# Autodesk Inventor assembly: 450LinearStage
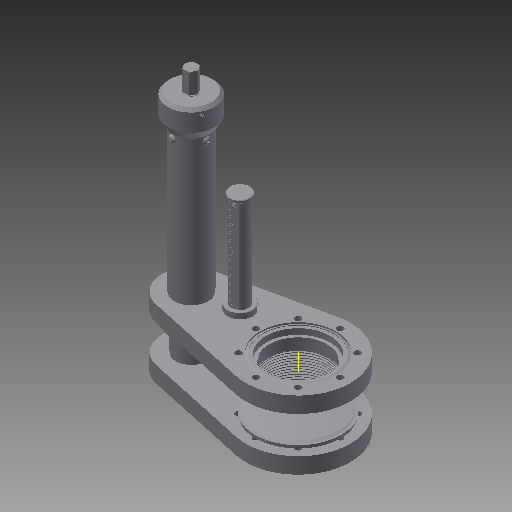
[picture p0: Inventor's stored thumbnail of the model, 512x512]
Saved by Autodesk Inventor 2018.1 (Build 221171000, 171)
## iProperties
Created: 2012-09-26
Part Number: 450LinearStage
Document SubType Name: Assembly
Designer: Sergey
Translation Standard: STEP AP203
FileName: 665524.STEP
PreProcessor: SolidWorks 2010
PostProcessor: Build: 236a, Release: 2009 RTM - Date: Fri 02/22/2008
Sent Units: Inches
Uncertainty: 1e-05
Author: Sergey
## Documents named in this file (23)
- C:\Users\michaels\Documents\SVN@Inventor\Moore Scienta DA30 system\450LinearStage.iam
- C:\Users\michaels\Documents\SVN@Inventor\Moore Scienta DA30 system\990985-04 Rev C-1-solid1.ipt
- C:\Users\michaels\Documents\SVN@Inventor\Moore Scienta DA30 system\990986-04 Rev B-1-solid1.ipt
- C:\Users\michaels\Documents\SVN@Inventor\Moore Scienta DA30 system\967848 Rev B-1-solid1.ipt
- C:\Users\michaels\Documents\SVN@Inventor\Moore Scienta DA30 system\966780 Rev --1-solid1.ipt
- C:\Users\michaels\Documents\SVN@Inventor\Moore Scienta DA30 system\966783-03 Rev G-1-solid1.ipt
- C:\Users\michaels\Documents\SVN@Inventor\Moore Scienta DA30 system\966782-03 Rev E-1-solid1.ipt
- C:\Users\michaels\Documents\SVN@Inventor\Moore Scienta DA30 system\990987-03 Rev A-1-solid1.ipt
- C:\Users\michaels\Documents\SVN@Inventor\Moore Scienta DA30 system\967830 Rev E-1-solid1.ipt
- C:\Users\michaels\Documents\SVN@Inventor\Moore Scienta DA30 system\966786 Rev A-1-solid1.ipt
- C:\Users\michaels\Documents\SVN@Inventor\Moore Scienta DA30 system\966787-07 Rev N-1_974032-07 Rev C-1-solid1.ipt
- C:\Users\michaels\Documents\SVN@Inventor\Moore Scienta DA30 system\966787-07 Rev N-1_974033-05 Rev B-1-solid1.ipt
- C:\Users\michaels\Documents\SVN@Inventor\Moore Scienta DA30 system\967874 Rev A-1-solid1.ipt
- C:\Users\michaels\Documents\SVN@Inventor\Moore Scienta DA30 system\967874 Rev A-2-solid1.ipt
- C:\Users\michaels\Documents\SVN@Inventor\Moore Scienta DA30 system\471025-665524-comp-1-solid1.ipt
- C:\Users\michaels\Documents\SVN@Inventor\Moore Scienta DA30 system\967838 Rev B-1-solid1.ipt
- C:\Users\michaels\Documents\SVN@Inventor\Moore Scienta DA30 system\012003-665524-1-solid1.ipt
- C:\Users\michaels\Documents\SVN@Inventor\Moore Scienta DA30 system\019536-1-solid1.ipt
- C:\Users\michaels\Documents\SVN@Inventor\Moore Scienta DA30 system\019635(8-32X.25)-1-solid1.ipt
- C:\Users\michaels\Documents\SVN@Inventor\Moore Scienta DA30 system\019635(8-32X.25)-2-solid1.ipt
- C:\Users\michaels\Documents\SVN@Inventor\Moore Scienta DA30 system\019635(8-32X.25)-3-solid1.ipt
- C:\Users\michaels\Documents\SVN@Inventor\Moore Scienta DA30 system\019635(8-32X.25)-4-solid1.ipt
- C:\Users\michaels\Documents\SVN@Inventor\Moore Scienta DA30 system\019307-1-solid1.ipt
## Components (22 placed, 22 different names)
1. 990985-04 Rev C-1-solid1:1 — Mate:2
2. 990986-04 Rev B-1-solid1:1
3. 967848 Rev B-1-solid1:1
4. 966780 Rev --1-solid1:1
5. 966783-03 Rev G-1-solid1:1
6. 966782-03 Rev E-1-solid1:1
7. 990987-03 Rev A-1-solid1:1 — Mate:1
8. 967830 Rev E-1-solid1:1
9. 966786 Rev A-1-solid1:1
10. 966787-07 Rev N-1_974032-07 Rev C-1-solid1:1
11. 966787-07 Rev N-1_974033-05 Rev B-1-solid1:1
12. 967874 Rev A-1-solid1:1
13. 967874 Rev A-2-solid1:1
14. 471025-665524-comp-1-solid1:1
15. 967838 Rev B-1-solid1:1
16. 012003-665524-1-solid1:1
17. 019536-1-solid1:1
18. 019635(8-32X.25)-1-solid1:1
19. 019635(8-32X.25)-2-solid1:1
20. 019635(8-32X.25)-3-solid1:1
21. 019635(8-32X.25)-4-solid1:1
22. 019307-1-solid1:1
## Relationships (2: Mate 2)
- Mate:1: 990987-03 Rev A-1-solid1:1
- Mate:2: 990985-04 Rev C-1-solid1:1
